# Autodesk Inventor assembly: Linear actuator assem 1
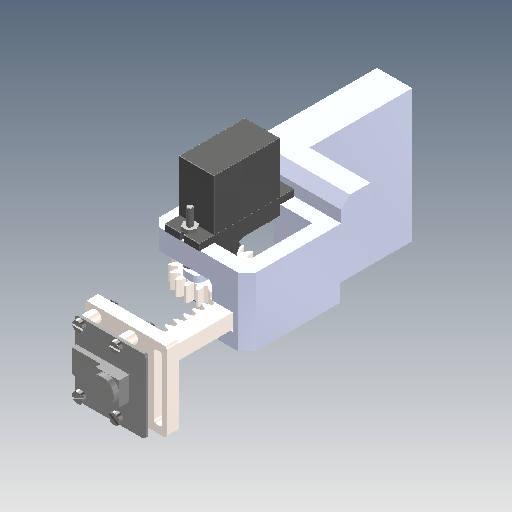
[picture p0: Inventor's stored thumbnail of the model, 512x512]
Saved by Autodesk Inventor 2020 (Build 240168000, 168)
## iProperties
Created: 2020-06-20
Part Number: Linear actuator assem 1
Document SubType Name: Assembly
Designer: ferrerx
Sending System: SolidWorks 2018
Last Author: ferrerx
Last Saved: 2020-06-26
Author: ferrerx
## Documents named in this file (12)
- C:\Users\ferrerx\Desktop\Projects\Prieto-Godino Lab\Drosophila Larvae Behavioural Device\Device design V3\Documentation\Mechanical components\Design files (Step and Autodesk inventor)\Inventor Assembly\Linear actuator assem 1.iam
- C:\Users\ferrerx\Desktop\Projects\Prieto-Godino Lab\Drosophila Larvae Behavioural Device\Device design V3\Documentation\Mechanical components\Design files (Step and Autodesk inventor)\Inventor Assembly\ISO - Spur gear 1M 20T 20PA 5FW ---S20A75H50L5.0N.ipt
- C:\Users\ferrerx\Desktop\Projects\Prieto-Godino Lab\Drosophila Larvae Behavioural Device\Device design V3\Documentation\Mechanical components\Design files (Step and Autodesk inventor)\Inventor Assembly\Linear actuator servo attachment.ipt
- C:\Users\ferrerx\Desktop\Projects\Prieto-Godino Lab\Drosophila Larvae Behavioural Device\Device design V3\Documentation\Mechanical components\Design files (Step and Autodesk inventor)\Inventor Assembly\MG90s_servo.ipt
- C:\Users\ferrerx\Desktop\Projects\Prieto-Godino Lab\Drosophila Larvae Behavioural Device\Device design V3\Documentation\Mechanical components\Design files (Step and Autodesk inventor)\Inventor Assembly\Servo lever.ipt
- C:\Users\ferrerx\Desktop\Projects\Prieto-Godino Lab\Drosophila Larvae Behavioural Device\Device design V3\Inventor Assembly\ISO - Rack-spur - rectangular 1M 20PA 5FW 5PH 125L---SAll.ipt
- C:\Users\ferrerx\Desktop\Projects\Prieto-Godino Lab\Drosophila Larvae Behavioural Device\Device design V3\Documentation\Mechanical components\Design files (Step and Autodesk inventor)\Inventor Assembly\pi_camera.ipt
- C:\Users\ferrerx\Documents\Inventor\Content Center Files\R2020\en-US\BS 4183(1)\BS 4183 - M2(1).ipt
- C:\Users\ferrerx\Documents\Inventor\Content Center Files\R2020\en-US\AS 1427(10)\AS 1427 - M2 x 16(7).ipt
- C:\Users\ferrerx\Documents\Inventor\Content Center Files\R2020\en-US\AS 1427(10)\AS 1427 - M2 x 12(7).ipt
- C:\Users\ferrerx\Documents\Inventor\Content Center Files\R2020\en-US\AS 1427(10)\AS 1427 - M2 x 4(7).ipt
- C:\Users\ferrerx\Documents\Inventor\Content Center Files\R2020\en-US\AS 1427(10)\AS 1427 - M2 x 10(7).ipt
## Components (21 placed, 11 different names)
1. ISO - Spur gear 1M 20T 20PA 5FW ---S20A75H50L5.0N:1 — Mate:25, Mate:26, Flush:2, Mate:35, Mate:36, Mate:39
2. Linear actuator servo attachment:1 — Mate:20, Mate:21, Flush:1, Mate:22, Mate:27, Mate:28, Mate:29, Mate:30
3. MG90s_servo:1 — Mate:21, Flush:1, Mate:22, Mate:23, Mate:24, Mate:33, Mate:34
4. Servo lever:1 — Mate:23, Mate:24, Mate:25, Mate:26, Mate:40
5. ISO - Rack-spur - rectangular 1M 20PA 5FW 5PH 125L---SAll:1 — Mate:1, Mate:2, Mate:3, Mate:4, Mate:5, Mate:6, Mate:7, Mate:16, Mate:17, Mate:18, Mate:19, Mate:20, Flush:2
6. pi_camera:1 — Mate:1, Mate:2, Mate:3, Mate:8, Mate:9, Mate:10, Mate:11
7. BS 4183 - Metric M2:1 — Mate:32, Mate:34
8. BS 4183 - Metric M2:2 — Mate:31, Mate:33
9. BS 4183 - Metric M2:3 — Mate:15, Mate:19
10. BS 4183 - Metric M2:4 — Mate:14, Mate:18
11. AS 1427 (8) - Metric M2 x 12:1 — Mate:4, Mate:9, Mate:14
12. AS 1427 (8) - Metric M2 x 12:3 — Mate:6, Mate:11, Mate:13
13. AS 1427 (8) - Metric M2 x 12:2 — Mate:5, Mate:10, Mate:12
14. AS 1427 (8) - Metric M2 x 12:4 — Mate:7, Mate:8, Mate:15
15. AS 1427 (8) - Metric M2 x 16:5 — Mate:28, Mate:30, Mate:31
16. AS 1427 (8) - Metric M2 x 16:6 — Mate:27, Mate:29, Mate:32
17. BS 4183 - Metric M2:5 — Mate:13, Mate:17
18. BS 4183 - Metric M2:6 — Mate:12, Mate:16
19. AS 1427 (8) - Metric M2 x 10:2 — Mate:35
20. AS 1427 (8) - Metric M2 x 10:1 — Mate:36
21. AS 1427 (8) - Metric M2 x 4:3 — Mate:39, Mate:40
## Relationships (40: Mate 38, Flush 2)
- Mate:1: ISO - Rack-spur - rectangular 1M 20PA 5FW 5PH 125L---SAll:1 ↔ pi_camera:1
- Mate:2: ISO - Rack-spur - rectangular 1M 20PA 5FW 5PH 125L---SAll:1 ↔ pi_camera:1
- Mate:3: ISO - Rack-spur - rectangular 1M 20PA 5FW 5PH 125L---SAll:1 ↔ pi_camera:1
- Mate:4: ISO - Rack-spur - rectangular 1M 20PA 5FW 5PH 125L---SAll:1 ↔ AS 1427 (8) - Metric M2 x 12:1
- Mate:5: ISO - Rack-spur - rectangular 1M 20PA 5FW 5PH 125L---SAll:1 ↔ AS 1427 (8) - Metric M2 x 12:2
- Mate:6: ISO - Rack-spur - rectangular 1M 20PA 5FW 5PH 125L---SAll:1 ↔ AS 1427 (8) - Metric M2 x 12:3
- Mate:7: ISO - Rack-spur - rectangular 1M 20PA 5FW 5PH 125L---SAll:1 ↔ AS 1427 (8) - Metric M2 x 12:4
- Mate:8: pi_camera:1 ↔ AS 1427 (8) - Metric M2 x 12:4
- Mate:9: pi_camera:1 ↔ AS 1427 (8) - Metric M2 x 12:1
- Mate:10: pi_camera:1 ↔ AS 1427 (8) - Metric M2 x 12:2
- Mate:11: pi_camera:1 ↔ AS 1427 (8) - Metric M2 x 12:3
- Mate:12: AS 1427 (8) - Metric M2 x 12:2 ↔ BS 4183 - Metric M2:6
- Mate:13: AS 1427 (8) - Metric M2 x 12:3 ↔ BS 4183 - Metric M2:5
- Mate:14: BS 4183 - Metric M2:4 ↔ AS 1427 (8) - Metric M2 x 12:1
- Mate:15: BS 4183 - Metric M2:3 ↔ AS 1427 (8) - Metric M2 x 12:4
- Mate:16: ISO - Rack-spur - rectangular 1M 20PA 5FW 5PH 125L---SAll:1 ↔ BS 4183 - Metric M2:6
- Mate:17: ISO - Rack-spur - rectangular 1M 20PA 5FW 5PH 125L---SAll:1 ↔ BS 4183 - Metric M2:5
- Mate:18: ISO - Rack-spur - rectangular 1M 20PA 5FW 5PH 125L---SAll:1 ↔ BS 4183 - Metric M2:4
- Mate:19: ISO - Rack-spur - rectangular 1M 20PA 5FW 5PH 125L---SAll:1 ↔ BS 4183 - Metric M2:3
- Mate:20: Linear actuator servo attachment:1 ↔ ISO - Rack-spur - rectangular 1M 20PA 5FW 5PH 125L---SAll:1
- Mate:21: Linear actuator servo attachment:1 ↔ MG90s_servo:1
- Flush:1 (5 mm): Linear actuator servo attachment:1 ↔ MG90s_servo:1
- Mate:22: Linear actuator servo attachment:1 ↔ MG90s_servo:1
- Mate:23: MG90s_servo:1 ↔ Servo lever:1
- Mate:24 (1 mm): MG90s_servo:1 ↔ Servo lever:1
- Mate:25: ISO - Spur gear 1M 20T 20PA 5FW ---S20A75H50L5.0N:1 ↔ Servo lever:1
- Mate:26: ISO - Spur gear 1M 20T 20PA 5FW ---S20A75H50L5.0N:1 ↔ Servo lever:1
- Mate:27: Linear actuator servo attachment:1 ↔ AS 1427 (8) - Metric M2 x 16:6
- Mate:28: Linear actuator servo attachment:1 ↔ AS 1427 (8) - Metric M2 x 16:5
- Mate:29: Linear actuator servo attachment:1 ↔ AS 1427 (8) - Metric M2 x 16:6
- Mate:30: Linear actuator servo attachment:1 ↔ AS 1427 (8) - Metric M2 x 16:5
- Mate:31: BS 4183 - Metric M2:2 ↔ AS 1427 (8) - Metric M2 x 16:5
- Mate:32: BS 4183 - Metric M2:1 ↔ AS 1427 (8) - Metric M2 x 16:6
- Mate:33: MG90s_servo:1 ↔ BS 4183 - Metric M2:2
- Mate:34: MG90s_servo:1 ↔ BS 4183 - Metric M2:1
- Flush:2: ISO - Spur gear 1M 20T 20PA 5FW ---S20A75H50L5.0N:1 ↔ ISO - Rack-spur - rectangular 1M 20PA 5FW 5PH 125L---SAll:1
- Mate:35: ISO - Spur gear 1M 20T 20PA 5FW ---S20A75H50L5.0N:1 ↔ AS 1427 (8) - Metric M2 x 10:2
- Mate:36: ISO - Spur gear 1M 20T 20PA 5FW ---S20A75H50L5.0N:1 ↔ AS 1427 (8) - Metric M2 x 10:1
- Mate:39: ISO - Spur gear 1M 20T 20PA 5FW ---S20A75H50L5.0N:1 ↔ AS 1427 (8) - Metric M2 x 4:3
- Mate:40: Servo lever:1 ↔ AS 1427 (8) - Metric M2 x 4:3
